# Autodesk Inventor assembly: Assembly1
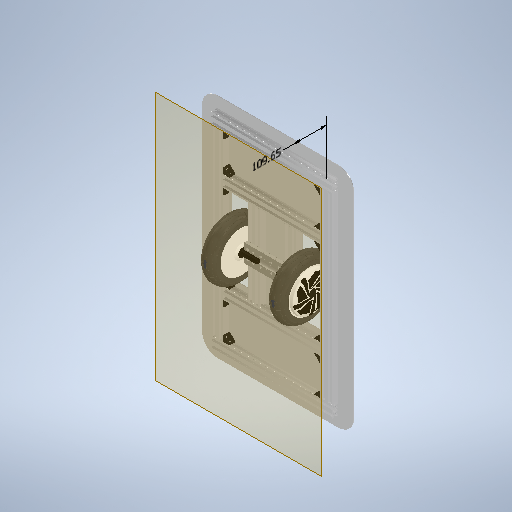
[picture p0: Inventor's stored thumbnail of the model, 512x512]
Saved by Autodesk Inventor 2025 (Build 290162000, 162)
## iProperties
Created: 2025-09-29
Part Number: Assembly1
Document SubType Name: Assembly
Designer: hp
Mass: 4352.41 g
Surface Area: 16168.4 cm^2
Volume: 1611.69 cm^3
Density: 2.70052 g/cm^3
Author: hp
## Documents named in this file (16)
- D:\gp amr\Assembly1.iam
- D:\gp amr\aluminum-extrusion-beams-1.snapshot.4\2040 - V-Slot\2040 - V-Slot.ipt
- D:\gp amr\corner-brackets-2.snapshot.2\OB-Bracket 2020\OB-Bracket 2020.ipt
- D:\gp amr\nut-m4-2020-10-6mm-1.snapshot.6\Nut-M4-2020\Nut-M4-2020.ipt
- C:\Users\hp\OneDrive - Faculty of Engineering Ain Shams University\Documents\Inventor\Content Center Files\R2025\en-US\ANSI B18.3.1M(2)\ANSI B18.3.1M - M4x0.7 x 8(6).ipt
- D:\gp amr\nut-m4-2020-10-6mm-1.snapshot.6\2040 - V-Slot.ipt 60.ipt
- D:\gp amr\aluminum-extrusion-beams-1.snapshot.4\2040 - V-Slot\2040 - V-Slot.ipt 320.ipt
- D:\gp amr\plate2mm.ipt
- C:\Users\hp\Downloads\hoverboard-wheel-8-bldc-motor-1.snapshot.4\Motor, BLDC, Hoverboard Wheel, 8.0in\Motor, BLDC, Hoverboard Wheel, 8.0in.ipt
- D:\gp amr\aluminum-extrusion-beams-1.snapshot.4\2040 - V-Slot\2040 - V-Slot.ipt 280.ipt
- C:\Users\hp\Downloads\hoverboard-wheel-8-bldc-motor-1.snapshot.4\hub_motor_mount_v19.ipt
- D:\gp amr\Assembly1\AIP\FEA\f78c4d0io.fins
- D:\gp amr\Assembly1\AIP\FEA\f78c4d0io.fsat
- D:\gp amr\Assembly1\AIP\FEA\f78c4d0io.ftes
- D:\gp amr\Assembly1\AIP\FEA\f78c4d0io.fwiz
- D:\gp amr\Assembly1\AIP\FEA\f78c4d0ow.fmsh
## Components (27 placed, 10 different names)
1. 2040 - V-Slot:1 — Mate:4, Flush:2, Mate:5, Mate:6, Mate:7, Mate:8, Flush:3, Mate:9, Flush:4, Mate:15, Angle:5, Flush:20, Mate:42
2. 2040 - V-Slot:4 — Mate:11, Mate:12, Flush:5, Mate:17, Mate:19, Mate:21
3. OB-Bracket 2020:1 — Mate:4, Flush:2, Insert:1, Insert:2, Mate:41
4. OB-Bracket 2020:2 — Mate:15, Mate:16, Flush:8
5. OB-Bracket 2020:3 — Mate:19, Mate:20, Flush:10
6. OB-Bracket 2020:4 — Mate:31, Mate:32, Flush:15
7. OB-Bracket 2020:5 — Mate:17, Mate:18, Flush:9
8. OB-Bracket 2020:6 — Mate:23, Mate:24, Flush:11
9. OB-Bracket 2020:7 — Mate:25, Mate:26, Flush:12
10. Nut-M4-2020:5 — Mate:5, Mate:6, Insert:1
11. Drilled Broached Hexagon Socket Head Cap Screw - 2 Holes - Metric M4x0.7 x 8:1 — Insert:2
12. 2040 - V-Slot.ipt 60:1 — Mate:7, Mate:8, Flush:3, Mate:13, Angle:2, Flush:6, Mate:14, Angle:3, Flush:7, Mate:18, Flush:9, Mate:28, Flush:13, Mate:30, Flush:14, Mate:36, Mate:37, Mate:41, Mate:44
13. 2040 - V-Slot.ipt 60:2 — Mate:9, Flush:4, Mate:11, Mate:12, Flush:5, Mate:16, Flush:8, Mate:20, Flush:10, Mate:24, Mate:26, Mate:32, Flush:15, Mate:34, Flush:16, Mate:39, Angle:4, Flush:19, Mate:40, Mate:47
14. 2040 - V-Slot.ipt 320:1 — Mate:13, Angle:2, Flush:6, Mate:22, Mate:25, Flush:12, Mate:29, Mate:31, Mate:35, Flush:17, Mate:39, Mate:42, Mate:45, Mate:48
15. 2040 - V-Slot.ipt 320:2 — Mate:14, Angle:3, Flush:7, Mate:21, Mate:22, Mate:23, Flush:11, Mate:27, Mate:33, Mate:38, Flush:18, Mate:50, Mate:52
16. OB-Bracket 2020:8 — Mate:27, Mate:28, Flush:13
17. OB-Bracket 2020:9 — Mate:29, Mate:30, Flush:14
18. OB-Bracket 2020:10 — Mate:33, Mate:34, Flush:16
19. OB-Bracket 2020:11 — Mate:35, Mate:36, Flush:17
20. OB-Bracket 2020:12 — Mate:37, Mate:38, Flush:18
21. plate2mm:1 — Angle:4, Angle:5, Flush:19, Mate:40, Flush:20, Flush:21, Flush:22, Mate:43, Mate:46, Angle:6
22. Motor, BLDC, Hoverboard Wheel, 8.0in:1 — Insert:3, Mate:53
23. Motor, BLDC, Hoverboard Wheel, 8.0in:2 — Insert:4
24. 2040 - V-Slot.ipt 280:1 — Mate:43, Mate:44, Mate:45, Mate:51, Flush:25
25. 2040 - V-Slot.ipt 280:2 — Mate:46, Mate:47, Mate:48, Mate:49, Flush:23
26. hub_motor_mount_v19:1 — Mate:49, Mate:50, Flush:23, Insert:3
27. hub_motor_mount_v19:2 — Mate:51, Mate:52, Insert:4, Flush:25
## Relationships (81: Mate 49, Flush 23, Angle 5, Insert 4)
- Mate:4: 2040 - V-Slot:1 ↔ OB-Bracket 2020:1
- Flush:2: 2040 - V-Slot:1 ↔ OB-Bracket 2020:1
- Mate:5: 2040 - V-Slot:1 ↔ Nut-M4-2020:5
- Mate:6: 2040 - V-Slot:1 ↔ Nut-M4-2020:5
- Insert:1 (0.57 mm): OB-Bracket 2020:1 ↔ Nut-M4-2020:5
- Insert:2: OB-Bracket 2020:1 ↔ Drilled Broached Hexagon Socket Head Cap Screw - 2 Holes - Metric M4x0.7 x 8:1
- Mate:7: 2040 - V-Slot:1 ↔ 2040 - V-Slot.ipt 60:1
- Mate:8: 2040 - V-Slot:1 ↔ 2040 - V-Slot.ipt 60:1
- Flush:3: 2040 - V-Slot:1 ↔ 2040 - V-Slot.ipt 60:1
- Mate:9: 2040 - V-Slot:1 ↔ 2040 - V-Slot.ipt 60:2
- Flush:4: 2040 - V-Slot:1 ↔ 2040 - V-Slot.ipt 60:2
- Mate:11: 2040 - V-Slot:4 ↔ 2040 - V-Slot.ipt 60:2
- Mate:12: 2040 - V-Slot:4 ↔ 2040 - V-Slot.ipt 60:2
- Flush:5: 2040 - V-Slot:4 ↔ 2040 - V-Slot.ipt 60:2
- Mate:13: 2040 - V-Slot.ipt 60:1 ↔ 2040 - V-Slot.ipt 320:1
- Angle:2 (0 deg): 2040 - V-Slot.ipt 60:1 ↔ 2040 - V-Slot.ipt 320:1
- Flush:6: 2040 - V-Slot.ipt 60:1 ↔ 2040 - V-Slot.ipt 320:1
- Mate:14: 2040 - V-Slot.ipt 60:1 ↔ 2040 - V-Slot.ipt 320:2
- Angle:3 (0 deg): 2040 - V-Slot.ipt 60:1 ↔ 2040 - V-Slot.ipt 320:2
- Flush:7: 2040 - V-Slot.ipt 60:1 ↔ 2040 - V-Slot.ipt 320:2
- Mate:15: 2040 - V-Slot:1 ↔ OB-Bracket 2020:2
- Mate:16: OB-Bracket 2020:2 ↔ 2040 - V-Slot.ipt 60:2
- Flush:8: OB-Bracket 2020:2 ↔ 2040 - V-Slot.ipt 60:2
- Mate:17: 2040 - V-Slot:4 ↔ OB-Bracket 2020:5
- Mate:18: OB-Bracket 2020:5 ↔ 2040 - V-Slot.ipt 60:1
- Flush:9: OB-Bracket 2020:5 ↔ 2040 - V-Slot.ipt 60:1
- Mate:19: 2040 - V-Slot:4 ↔ OB-Bracket 2020:3
- Mate:20: OB-Bracket 2020:3 ↔ 2040 - V-Slot.ipt 60:2
- Flush:10: OB-Bracket 2020:3 ↔ 2040 - V-Slot.ipt 60:2
- Mate:21 (120 mm): 2040 - V-Slot:4 ↔ 2040 - V-Slot.ipt 320:2
- Mate:22 (280 mm): 2040 - V-Slot.ipt 320:1 ↔ 2040 - V-Slot.ipt 320:2
- Mate:23: OB-Bracket 2020:6 ↔ 2040 - V-Slot.ipt 320:2
- Mate:24: OB-Bracket 2020:6 ↔ 2040 - V-Slot.ipt 60:2
- Flush:11: OB-Bracket 2020:6 ↔ 2040 - V-Slot.ipt 320:2
- Mate:25: OB-Bracket 2020:7 ↔ 2040 - V-Slot.ipt 320:1
- Mate:26: OB-Bracket 2020:7 ↔ 2040 - V-Slot.ipt 60:2
- Flush:12: OB-Bracket 2020:7 ↔ 2040 - V-Slot.ipt 320:1
- Mate:27: 2040 - V-Slot.ipt 320:2 ↔ OB-Bracket 2020:8
- Mate:28: 2040 - V-Slot.ipt 60:1 ↔ OB-Bracket 2020:8
- Flush:13: 2040 - V-Slot.ipt 60:1 ↔ OB-Bracket 2020:8
- Mate:29: 2040 - V-Slot.ipt 320:1 ↔ OB-Bracket 2020:9
- Mate:30: 2040 - V-Slot.ipt 60:1 ↔ OB-Bracket 2020:9
- Flush:14: 2040 - V-Slot.ipt 60:1 ↔ OB-Bracket 2020:9
- Mate:31: OB-Bracket 2020:4 ↔ 2040 - V-Slot.ipt 320:1
- Mate:32: OB-Bracket 2020:4 ↔ 2040 - V-Slot.ipt 60:2
- Flush:15: OB-Bracket 2020:4 ↔ 2040 - V-Slot.ipt 60:2
- Mate:33: 2040 - V-Slot.ipt 320:2 ↔ OB-Bracket 2020:10
- Mate:34: 2040 - V-Slot.ipt 60:2 ↔ OB-Bracket 2020:10
- Flush:16: 2040 - V-Slot.ipt 60:2 ↔ OB-Bracket 2020:10
- Mate:35: 2040 - V-Slot.ipt 320:1 ↔ OB-Bracket 2020:11
- Mate:36: 2040 - V-Slot.ipt 60:1 ↔ OB-Bracket 2020:11
- Flush:17: 2040 - V-Slot.ipt 320:1 ↔ OB-Bracket 2020:11
- Mate:37: 2040 - V-Slot.ipt 60:1 ↔ OB-Bracket 2020:12
- Mate:38: 2040 - V-Slot.ipt 320:2 ↔ OB-Bracket 2020:12
- Flush:18: 2040 - V-Slot.ipt 320:2 ↔ OB-Bracket 2020:12
- Mate:39: 2040 - V-Slot.ipt 60:2 ↔ 2040 - V-Slot.ipt 320:1
- Angle:4 (0 deg): 2040 - V-Slot.ipt 60:2 ↔ plate2mm:1
- Angle:5 (0 deg): 2040 - V-Slot:1 ↔ plate2mm:1
- Flush:19 (-50 mm): 2040 - V-Slot.ipt 60:2 ↔ plate2mm:1
- Mate:40: 2040 - V-Slot.ipt 60:2 ↔ plate2mm:1
- Flush:20 (35 mm): 2040 - V-Slot:1 ↔ plate2mm:1
- Mate:41: OB-Bracket 2020:1 ↔ 2040 - V-Slot.ipt 60:1
- Flush:21: plate2mm:1
- Flush:22: plate2mm:1
- Mate:42 (120 mm): 2040 - V-Slot:1 ↔ 2040 - V-Slot.ipt 320:1
- Mate:43: plate2mm:1 ↔ 2040 - V-Slot.ipt 280:1
- Mate:44 (80 mm): 2040 - V-Slot.ipt 60:1 ↔ 2040 - V-Slot.ipt 280:1
- Mate:45: 2040 - V-Slot.ipt 320:1 ↔ 2040 - V-Slot.ipt 280:1
- Mate:46: plate2mm:1 ↔ 2040 - V-Slot.ipt 280:2
- Mate:47 (80 mm): 2040 - V-Slot.ipt 60:2 ↔ 2040 - V-Slot.ipt 280:2
- Mate:48: 2040 - V-Slot.ipt 320:1 ↔ 2040 - V-Slot.ipt 280:2
- Mate:49: 2040 - V-Slot.ipt 280:2 ↔ hub_motor_mount_v19:1
- Mate:50 (110 mm): 2040 - V-Slot.ipt 320:2 ↔ hub_motor_mount_v19:1
- Flush:23: 2040 - V-Slot.ipt 280:2 ↔ hub_motor_mount_v19:1
- Mate:51: 2040 - V-Slot.ipt 280:1 ↔ hub_motor_mount_v19:2
- Mate:52 (110 mm): 2040 - V-Slot.ipt 320:2 ↔ hub_motor_mount_v19:2
- Insert:3: Motor, BLDC, Hoverboard Wheel, 8.0in:1 ↔ hub_motor_mount_v19:1
- Insert:4: Motor, BLDC, Hoverboard Wheel, 8.0in:2 ↔ hub_motor_mount_v19:2
- Flush:25: 2040 - V-Slot.ipt 280:1 ↔ hub_motor_mount_v19:2
- Mate:53: Motor, BLDC, Hoverboard Wheel, 8.0in:1
- Angle:6 (0 deg): plate2mm:1
## Named parameters: sa_0 = 100000
note: some values were not read from the file. Shown as the stored number, unit unknown: "sa_0".
